# Autodesk Inventor assembly: 付け根ロール_1
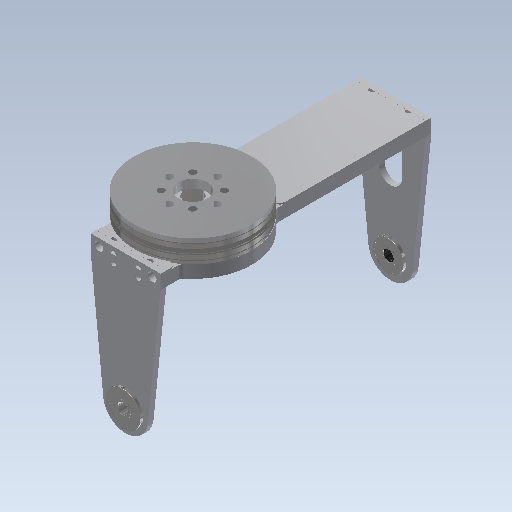
[picture p0: Inventor's stored thumbnail of the model, 512x512]
Saved by Autodesk Inventor 2020 (Build 240168000, 168)
## iProperties
Created: 2016-05-01
Part Number: 付け根ロール_1
Document SubType Name: Assembly
Designer: hiroaki
Mass: 38.2338 g
Surface Area: 222.3 cm^2
Volume: 16.8041 cm^3
Density: 2.27527 g/cm^3
Author: hiroaki
## Documents named in this file (10)
- C:\Users\Masato\Documents\Inventor\CIT Brains_Inventor\OpenPlatform_ver3_0\下半身_160823\付け根ロール\付け根ロール_1.iam
- C:\Users\Masato\Documents\Inventor\CIT Brains_Inventor\OpenPlatform_ver3_0\下半身_160823\付け根ロール\付け根ロール_メインフレーム_1_1.ipt
- C:\Users\Masato\Documents\Inventor\CIT Brains_Inventor\OpenPlatform_ver3_0\既製品\BA2542\core_BA2542.ipt
- C:\Users\Masato\Documents\Inventor\CIT Brains_Inventor\OpenPlatform_ver3_0\下半身_160823\付け根ロール\付け根ロール_サブフレーム_1_4.ipt
- C:\Users\Masato\Documents\Inventor\CIT Brains_Inventor\OpenPlatform_ver3_0\既製品\BA2542\washer_BA2542.ipt
- C:\Users\Masato\Documents\Inventor\CIT Brains_Inventor\OpenPlatform_ver3_0\既製品\MSU-306-03.ipt
- C:\Users\Masato\Documents\Inventor\CIT Brains_Inventor\OpenPlatform_ver3_0\下半身_160823\付け根ロール\付け根ロール_サブフレーム_6_5.ipt
- C:\Users\Masato\Documents\Inventor\CIT Brains_Inventor\OpenPlatform_ver3_0\下半身_160823\付け根ロール\付け根ロール_サブフレーム_6_6.ipt
- C:\Users\Masato\Documents\Inventor\CIT Brains_Inventor\OpenPlatform_ver3_0\既製品\NSK_RB_F694ZZ\F694ZZ.iam
- C:\Users\Masato\Documents\Inventor\CIT Brains_Inventor\OpenPlatform_ver3_0\下半身\リンク\スペーサ\付け根_スペーサ_1_2.ipt
## Components (14 placed, 9 different names)
1. 付け根ロール_メインフレーム_1_1:1 — 挿入:29, 挿入:31, 挿入:32, 挿入:33, 挿入:34, 挿入:38, 挿入:39, 挿入:40, 挿入:41
2. core_BA2542:1 — 挿入:30
3. core_BA2542:2 — 挿入:24
4. 付け根ロール_サブフレーム_1_4:1 — 挿入:24, 挿入:35, 挿入:36, 挿入:37
5. washer_BA2542:1 — 挿入:29, 挿入:30
6. MSU-306-03:1 — 挿入:31, 挿入:35
7. MSU-306-03:2 — 挿入:32, 挿入:36
8. MSU-306-03:3 — 挿入:33
9. MSU-306-03:4 — 挿入:34, 挿入:37
10. 付け根ロール_サブフレーム_6_5:1 — 挿入:40, 挿入:41, 挿入:42
11. 付け根ロール_サブフレーム_6_6:1 — 挿入:38, 挿入:39, 挿入:43
12. F694ZZ:1 [sub-assembly] — 挿入:42, 挿入:44
13. F694ZZ:2 [sub-assembly] — 挿入:43
14. 付け根_スペーサ_1_2:1 — 挿入:44
## Relationships (17: Insert 17)
- 挿入:24 [Insert]: core_BA2542:2 ↔ 付け根ロール_サブフレーム_1_4:1
- 挿入:29 [Insert]: 付け根ロール_メインフレーム_1_1:1 ↔ washer_BA2542:1
- 挿入:30 [Insert]: core_BA2542:1 ↔ washer_BA2542:1
- 挿入:31 [Insert]: 付け根ロール_メインフレーム_1_1:1 ↔ MSU-306-03:1
- 挿入:32 [Insert]: 付け根ロール_メインフレーム_1_1:1 ↔ MSU-306-03:2
- 挿入:33 [Insert]: 付け根ロール_メインフレーム_1_1:1 ↔ MSU-306-03:3
- 挿入:34 [Insert]: 付け根ロール_メインフレーム_1_1:1 ↔ MSU-306-03:4
- 挿入:35 [Insert]: 付け根ロール_サブフレーム_1_4:1 ↔ MSU-306-03:1
- 挿入:36 [Insert]: 付け根ロール_サブフレーム_1_4:1 ↔ MSU-306-03:2
- 挿入:37 [Insert]: 付け根ロール_サブフレーム_1_4:1 ↔ MSU-306-03:4
- 挿入:38 [Insert]: 付け根ロール_メインフレーム_1_1:1 ↔ 付け根ロール_サブフレーム_6_6:1
- 挿入:39 [Insert]: 付け根ロール_メインフレーム_1_1:1 ↔ 付け根ロール_サブフレーム_6_6:1
- 挿入:40 [Insert]: 付け根ロール_メインフレーム_1_1:1 ↔ 付け根ロール_サブフレーム_6_5:1
- 挿入:41 [Insert]: 付け根ロール_メインフレーム_1_1:1 ↔ 付け根ロール_サブフレーム_6_5:1
- 挿入:42 [Insert]: 付け根ロール_サブフレーム_6_5:1 ↔ F694ZZ:1
- 挿入:43 [Insert]: 付け根ロール_サブフレーム_6_6:1 ↔ F694ZZ:2
- 挿入:44 [Insert]: F694ZZ:1 ↔ 付け根_スペーサ_1_2:1
